# Autodesk Inventor assembly: esqMT
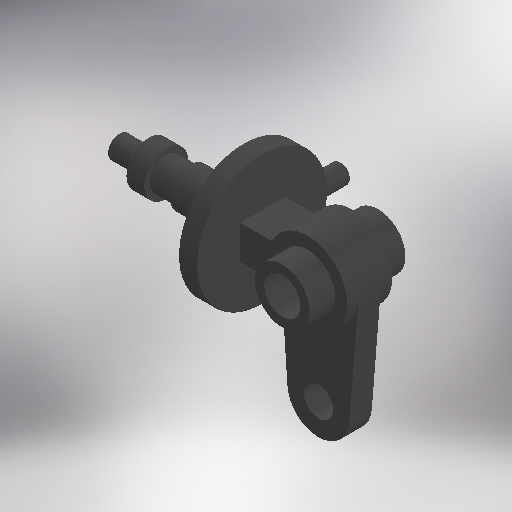
[picture p0: Inventor's stored thumbnail of the model, 512x512]
Saved by Autodesk Inventor 2025.3 (Build 293356000, 356)
## iProperties
Created: 2026-09-27
Part Number: esqMT
Document SubType Name: Assembly
Designer: user
Author: user
## Documents named in this file (3)
- C:\Users\user\Desktop\roda_camaro\esqMT.iam
- C:\Users\user\Desktop\roda_camaro\travainterna.ipt
- C:\Users\user\Desktop\roda_camaro\travaInternaRoda.ipt
## Components (2 placed, 2 different names)
1. travainterna:1 — Rígida:1
2. travaInternaRoda:1 — Rígida:1
## Relationships (1: WeldJoint 1)
- Rígida:1 [WeldJoint]: travainterna:1 ↔ travaInternaRoda:1
